# Autodesk Inventor assembly: RoomWallAssembly
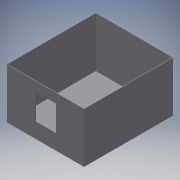
[picture p0: Inventor's stored thumbnail of the model, 180x180]
Saved by Autodesk Inventor 2018 (Build 220112000, 112)
## iProperties
Created: 2019-04-28
Part Number: RoomWallAssembly
Document SubType Name: Assembly
Designer: snipe
Author: snipe
## Documents named in this file (6)
- C:\Users\snipe\Documents\FrileyResidenceHallRoomCAD\4517\RoomWallAssembly.iam
- C:\Users\snipe\Documents\FrileyResidenceHallRoomCAD\4517\Footprint.ipt
- C:\Users\snipe\Documents\FrileyResidenceHallRoomCAD\4517\NorthWall.ipt
- C:\Users\snipe\Documents\FrileyResidenceHallRoomCAD\4517\SouthWall.ipt
- C:\Users\snipe\Documents\FrileyResidenceHallRoomCAD\4517\EastWall.ipt
- C:\Users\snipe\Documents\FrileyResidenceHallRoomCAD\4517\WestWall.ipt
## Components (5 placed, 5 different names)
1. Footprint:1 — Mate:1, Flush:1, Mate:4, Mate:3, Flush:2, Mate:5, Mate:6, Flush:3, Mate:7, Mate:8, Flush:4, Mate:9
2. NorthWall:1 — Mate:4, Mate:3, Flush:2
3. SouthWall:1 — Mate:1, Flush:1, Mate:7
4. EastWall:1 — Mate:5, Mate:6, Flush:3
5. WestWall:1 — Mate:8, Flush:4, Mate:9
## Relationships (12: Mate 8, Flush 4)
- Mate:1: Footprint:1 ↔ SouthWall:1
- Flush:1: Footprint:1 ↔ SouthWall:1
- Mate:4: Footprint:1 ↔ NorthWall:1
- Mate:3: Footprint:1 ↔ NorthWall:1
- Flush:2: Footprint:1 ↔ NorthWall:1
- Mate:5: Footprint:1 ↔ EastWall:1
- Mate:6: Footprint:1 ↔ EastWall:1
- Flush:3: Footprint:1 ↔ EastWall:1
- Mate:7: Footprint:1 ↔ SouthWall:1
- Mate:8: Footprint:1 ↔ WestWall:1
- Flush:4: Footprint:1 ↔ WestWall:1
- Mate:9: Footprint:1 ↔ WestWall:1
